# Autodesk Inventor assembly: 总装配
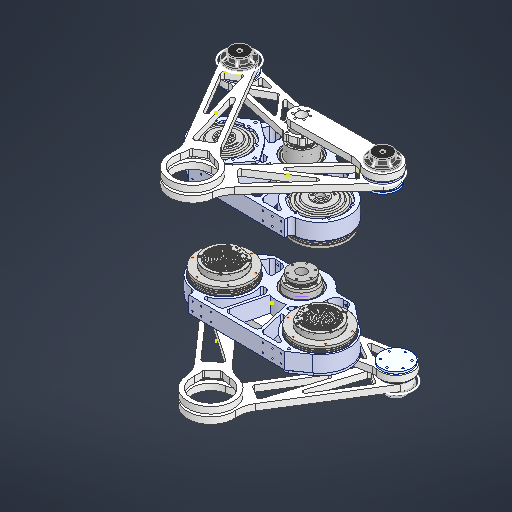
[picture p0: Inventor's stored thumbnail of the model, 512x512]
Saved by Autodesk Inventor 2025 (Build 290162000, 162)
## iProperties
Created: 2025-04-19
Part Number: 总装配
Document SubType Name: Assembly
Designer: XH
Author: XH
## Documents named in this file (2)
- C:\1A_Engineering_files\RCInventor并联腿\总装配.iam
- C:\1A_Engineering_files\RCInventor并联腿\装配体2.iam
## Components (2 placed, 1 different names)
1. 装配体2:1 [sub-assembly] — 表面齐平:1, 配合:1
2. 装配体2:2 [sub-assembly] — 表面齐平:1, 配合:1
## Relationships (2: Flush 1, Mate 1)
- 表面齐平:1 [Flush]: 装配体2:1 ↔ 装配体2:2
- 配合:1 [Mate]: 装配体2:1 ↔ 装配体2:2
